# Autodesk Inventor assembly: brazo
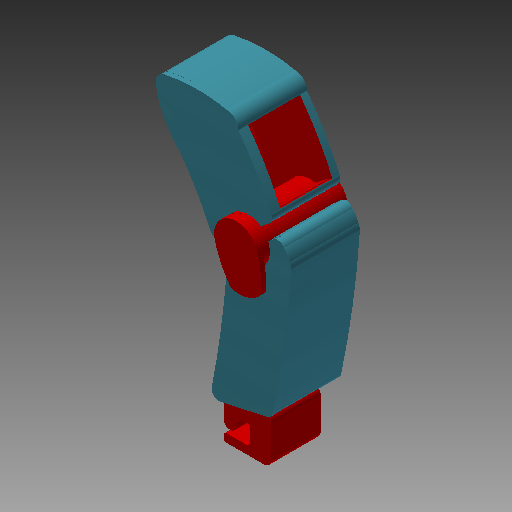
[picture p0: Inventor's stored thumbnail of the model, 512x512]
Saved by Autodesk Inventor 2019 (Build 230136000, 136)
## iProperties
Part Number: brazo
Material: Genérico
Document SubType Name: Assembly
Designer: Kevin
Author: Kevin
## Documents named in this file (6)
- D:\Documents\Kevin\robot\brazo.iam
- D:\Documents\Kevin\robot\brazos\brazoderech\brazoderecho.ipt
- D:\Documents\Kevin\robot\tapabrazo.ipt
- D:\Documents\Kevin\robot\tapabrazo2.ipt
- D:\Documents\Kevin\robot\codo.ipt
- D:\Documents\Kevin\robot\mano.ipt
## Components (7 placed, 5 different names)
1. brazoderecho:1 — Coincidencia:1, Coincidencia:2, De rotación:2, De rotación:3, Coincidencia:3, De rotación:4
2. tapabrazo:1 — Coincidencia:1
3. tapabrazo2:1 — Coincidencia:2
4. codo:2 — De rotación:2
5. codo:4 — De rotación:3
6. mano:1 — Coincidencia:3
7. tapabrazo:2 — De rotación:4
## Relationships (6: Mate 3, RevoluteJoint 3)
- Coincidencia:1 [Mate]: brazoderecho:1 ↔ tapabrazo:1
- Coincidencia:2 [Mate]: brazoderecho:1 ↔ tapabrazo2:1
- De rotación:2 [RevoluteJoint]: brazoderecho:1 ↔ codo:2
- De rotación:3 [RevoluteJoint]: brazoderecho:1 ↔ codo:4
- Coincidencia:3 [Mate]: brazoderecho:1 ↔ mano:1
- De rotación:4 [RevoluteJoint]: brazoderecho:1 ↔ tapabrazo:2
